# Autodesk Inventor assembly: Assembly1
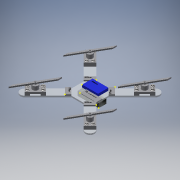
[picture p0: Inventor's stored thumbnail of the model, 180x180]
Saved by Autodesk Inventor 2019.4 (Build 234330000, 330)
## iProperties
Created: 2019-06-13
Part Number: Assembly1
Document SubType Name: Assembly
Designer: abdel
Author: abdel
## Documents named in this file (11)
- C:\Users\abdel\Downloads\10% project (laptop)-20190621T144919Z-001\10_ project (laptop)\drone\drone inventor\Assembly1.iam
- C:\Users\abdel\Downloads\10% project (laptop)-20190621T144919Z-001\10_ project (laptop)\drone\drone inventor\drone frame.ipt
- C:\Users\abdel\Downloads\10% project (laptop)-20190621T144919Z-001\10_ project (laptop)\drone\drone inventor\MotorController.ipt
- C:\Users\abdel\Downloads\10% project (laptop)-20190621T144919Z-001\10_ project (laptop)\drone\drone inventor\BracketOfTheBracket.ipt
- C:\Users\abdel\Downloads\10% project (laptop)-20190621T144919Z-001\10_ project (laptop)\drone\drone inventor\bracket for drone.ipt
- C:\Users\abdel\Downloads\10% project (laptop)-20190621T144919Z-001\10_ project (laptop)\drone\drone inventor\Motor.ipt
- C:\Users\abdel\Downloads\10% project (laptop)-20190621T144919Z-001\10_ project (laptop)\drone\drone inventor\Propeller.ipt
- C:\Users\abdel\Downloads\10% project (laptop)-20190621T144919Z-001\10_ project (laptop)\drone\drone inventor\battery.ipt
- C:\Users\abdel\Downloads\10% project (laptop)-20190621T144919Z-001\10_ project (laptop)\drone\drone inventor\GyroSensor.ipt
- C:\Users\abdel\Documents\Inventor\Content Center Files\R2019\en-US\GB_T 16674.1-2004\Bolt GB_T 16674.1 M8 x 16.ipt
- C:\Users\abdel\Downloads\10% project (laptop)-20190621T144919Z-001\10_ project (laptop)\drone\drone inventor\Arduino.ipt
## Components (44 placed, 10 different names)
1. battery:1 — Mate:41, Flush:24
2. bracket for drone:1 — Flush:3, Flush:4, Mate:4, Flush:5, Flush:6, Mate:5, Mate:6, Mate:7, Flush:11, Mate:42, Mate:43, Mate:44, Mate:45, Mate:46, Mate:47, Mate:48, Mate:49
3. drone frame:1 — Mate:12, Mate:13, Flush:11, Mate:18, Mate:19, Flush:16, Mate:24, Mate:25, Flush:21, Mate:26, Mate:27, Flush:22, Mate:28, Mate:29, Mate:30, Mate:31, Mate:32, Mate:33, Mate:34, Mate:35, Mate:36, Mate:37, Mate:38, Mate:39, Mate:40, Flush:23, Mate:41, Flush:24, Mate:66
4. Motor:1 — Rotational:1, Mate:6, Mate:7
5. MotorController:1 — Mate:28, Mate:29, Mate:30
6. Propeller:1 — Rotational:1
7. BracketOfTheBracket:3 — Flush:5, Flush:6, Mate:5
8. BracketOfTheBracket:5 — Flush:3, Flush:4, Mate:4, Mate:12, Mate:13
9. bracket for drone:2 — Flush:22, Mate:58, Mate:59, Mate:60, Mate:61, Mate:62, Mate:63, Mate:64, Mate:65
10. Motor:2
11. Propeller:2
12. BracketOfTheBracket:6
13. BracketOfTheBracket:7 — Mate:26, Mate:27
14. bracket for drone:3 — Flush:16, Mate:50, Mate:51, Mate:52, Mate:53, Mate:54, Mate:55, Mate:56, Mate:57
15. Motor:3
16. Propeller:3
17. BracketOfTheBracket:8
18. BracketOfTheBracket:9 — Mate:18, Mate:19
19. bracket for drone:4 — Flush:21, Insert:1, Insert:2, Insert:3, Insert:4
20. Motor:4
21. Propeller:4
22. BracketOfTheBracket:10 — Mate:25
23. BracketOfTheBracket:11 — Mate:24
24. MotorController:2 — Mate:31, Mate:32, Mate:33
25. MotorController:3 — Mate:34, Mate:35, Mate:36
26. MotorController:4 — Mate:37, Mate:38, Mate:39
27. GyroSensor:1 — Mate:40, Flush:23
28. Bolt GB/T 16674.1-2004 M8x16:1 — Insert:1
29. Bolt GB/T 16674.1-2004 M8x16:2 — Insert:2
30. Bolt GB/T 16674.1-2004 M8x16:3 — Insert:3
31. Bolt GB/T 16674.1-2004 M8x16:4 — Insert:4
32. Bolt GB/T 16674.1-2004 M8x16:5 — Mate:42, Mate:43
33. Bolt GB/T 16674.1-2004 M8x16:6 — Mate:44, Mate:45
34. Bolt GB/T 16674.1-2004 M8x16:7 — Mate:46, Mate:47
35. Bolt GB/T 16674.1-2004 M8x16:8 — Mate:48, Mate:49
36. Bolt GB/T 16674.1-2004 M8x16:9 — Mate:50, Mate:51
37. Bolt GB/T 16674.1-2004 M8x16:10 — Mate:52, Mate:53
38. Bolt GB/T 16674.1-2004 M8x16:11 — Mate:54, Mate:55
39. Bolt GB/T 16674.1-2004 M8x16:12 — Mate:56, Mate:57
40. Bolt GB/T 16674.1-2004 M8x16:13 — Mate:58, Mate:59
41. Bolt GB/T 16674.1-2004 M8x16:14 — Mate:60, Mate:61
42. Bolt GB/T 16674.1-2004 M8x16:15 — Mate:62, Mate:63
43. Bolt GB/T 16674.1-2004 M8x16:16 — Mate:64, Mate:65
44. Arduino:1 — Mate:66
## Relationships (93: Mate 63, Flush 22, RevoluteJoint 4, Insert 4)
- Rotational:1 [RevoluteJoint]: Motor:1 ↔ Propeller:1
- Flush:3: bracket for drone:1 ↔ BracketOfTheBracket:5
- Flush:4: bracket for drone:1 ↔ BracketOfTheBracket:5
- Mate:4: bracket for drone:1 ↔ BracketOfTheBracket:5
- Flush:5: bracket for drone:1 ↔ BracketOfTheBracket:3
- Flush:6: bracket for drone:1 ↔ BracketOfTheBracket:3
- Mate:5: bracket for drone:1 ↔ BracketOfTheBracket:3
- Mate:6: bracket for drone:1 ↔ Motor:1
- Mate:7: bracket for drone:1 ↔ Motor:1
- [RevoluteJoint]: Motor:2 ↔ Propeller:2
- [Flush]: bracket for drone:2 ↔ BracketOfTheBracket:7
- [Flush]: bracket for drone:2 ↔ BracketOfTheBracket:7
- [Mate]: bracket for drone:2 ↔ BracketOfTheBracket:7
- [Flush]: bracket for drone:2 ↔ BracketOfTheBracket:6
- [Flush]: bracket for drone:2 ↔ BracketOfTheBracket:6
- [Mate]: bracket for drone:2 ↔ BracketOfTheBracket:6
- [Mate]: bracket for drone:2 ↔ Motor:2
- [Mate]: bracket for drone:2 ↔ Motor:2
- Mate:12: drone frame:1 ↔ BracketOfTheBracket:5
- Mate:13: drone frame:1 ↔ BracketOfTheBracket:5
- Flush:11: bracket for drone:1 ↔ drone frame:1
- [RevoluteJoint]: Motor:3 ↔ Propeller:3
- [Flush]: bracket for drone:3 ↔ BracketOfTheBracket:9
- [Flush]: bracket for drone:3 ↔ BracketOfTheBracket:9
- [Mate]: bracket for drone:3 ↔ BracketOfTheBracket:9
- [Flush]: bracket for drone:3 ↔ BracketOfTheBracket:8
- [Flush]: bracket for drone:3 ↔ BracketOfTheBracket:8
- [Mate]: bracket for drone:3 ↔ BracketOfTheBracket:8
- [Mate]: bracket for drone:3 ↔ Motor:3
- [Mate]: bracket for drone:3 ↔ Motor:3
- Mate:18: drone frame:1 ↔ BracketOfTheBracket:9
- Mate:19: drone frame:1 ↔ BracketOfTheBracket:9
- Flush:16: drone frame:1 ↔ bracket for drone:3
- [RevoluteJoint]: Motor:4 ↔ Propeller:4
- [Flush]: bracket for drone:4 ↔ BracketOfTheBracket:11
- [Flush]: bracket for drone:4 ↔ BracketOfTheBracket:11
- [Mate]: bracket for drone:4 ↔ BracketOfTheBracket:11
- [Flush]: bracket for drone:4 ↔ BracketOfTheBracket:10
- [Flush]: bracket for drone:4 ↔ BracketOfTheBracket:10
- [Mate]: bracket for drone:4 ↔ BracketOfTheBracket:10
- [Mate]: bracket for drone:4 ↔ Motor:4
- [Mate]: bracket for drone:4 ↔ Motor:4
- Mate:24: drone frame:1 ↔ BracketOfTheBracket:11
- Mate:25: drone frame:1 ↔ BracketOfTheBracket:10
- Flush:21: drone frame:1 ↔ bracket for drone:4
- Mate:26: drone frame:1 ↔ BracketOfTheBracket:7
- Mate:27: drone frame:1 ↔ BracketOfTheBracket:7
- Flush:22: drone frame:1 ↔ bracket for drone:2
- Mate:28: drone frame:1 ↔ MotorController:1
- Mate:29: drone frame:1 ↔ MotorController:1
- Mate:30: drone frame:1 ↔ MotorController:1
- Mate:31: drone frame:1 ↔ MotorController:2
- Mate:32: drone frame:1 ↔ MotorController:2
- Mate:33: drone frame:1 ↔ MotorController:2
- Mate:34: drone frame:1 ↔ MotorController:3
- Mate:35: drone frame:1 ↔ MotorController:3
- Mate:36: drone frame:1 ↔ MotorController:3
- Mate:37: drone frame:1 ↔ MotorController:4
- Mate:38: drone frame:1 ↔ MotorController:4
- Mate:39: drone frame:1 ↔ MotorController:4
- Mate:40: drone frame:1 ↔ GyroSensor:1
- Flush:23: drone frame:1 ↔ GyroSensor:1
- Mate:41: battery:1 ↔ drone frame:1
- Flush:24: battery:1 ↔ drone frame:1
- Insert:1: bracket for drone:4 ↔ Bolt GB/T 16674.1-2004 M8x16:1
- Insert:2: bracket for drone:4 ↔ Bolt GB/T 16674.1-2004 M8x16:2
- Insert:3: bracket for drone:4 ↔ Bolt GB/T 16674.1-2004 M8x16:3
- Insert:4: bracket for drone:4 ↔ Bolt GB/T 16674.1-2004 M8x16:4
- Mate:42: bracket for drone:1 ↔ Bolt GB/T 16674.1-2004 M8x16:5
- Mate:43: bracket for drone:1 ↔ Bolt GB/T 16674.1-2004 M8x16:5
- Mate:44: bracket for drone:1 ↔ Bolt GB/T 16674.1-2004 M8x16:6
- Mate:45: bracket for drone:1 ↔ Bolt GB/T 16674.1-2004 M8x16:6
- Mate:46: bracket for drone:1 ↔ Bolt GB/T 16674.1-2004 M8x16:7
- Mate:47: bracket for drone:1 ↔ Bolt GB/T 16674.1-2004 M8x16:7
- Mate:48: bracket for drone:1 ↔ Bolt GB/T 16674.1-2004 M8x16:8
- Mate:49: bracket for drone:1 ↔ Bolt GB/T 16674.1-2004 M8x16:8
- Mate:50: bracket for drone:3 ↔ Bolt GB/T 16674.1-2004 M8x16:9
- Mate:51: bracket for drone:3 ↔ Bolt GB/T 16674.1-2004 M8x16:9
- Mate:52: bracket for drone:3 ↔ Bolt GB/T 16674.1-2004 M8x16:10
- Mate:53: bracket for drone:3 ↔ Bolt GB/T 16674.1-2004 M8x16:10
- Mate:54: bracket for drone:3 ↔ Bolt GB/T 16674.1-2004 M8x16:11
- Mate:55: bracket for drone:3 ↔ Bolt GB/T 16674.1-2004 M8x16:11
- Mate:56: bracket for drone:3 ↔ Bolt GB/T 16674.1-2004 M8x16:12
- Mate:57: bracket for drone:3 ↔ Bolt GB/T 16674.1-2004 M8x16:12
- Mate:58: bracket for drone:2 ↔ Bolt GB/T 16674.1-2004 M8x16:13
- Mate:59: bracket for drone:2 ↔ Bolt GB/T 16674.1-2004 M8x16:13
- Mate:60: bracket for drone:2 ↔ Bolt GB/T 16674.1-2004 M8x16:14
- Mate:61: bracket for drone:2 ↔ Bolt GB/T 16674.1-2004 M8x16:14
- Mate:62: bracket for drone:2 ↔ Bolt GB/T 16674.1-2004 M8x16:15
- Mate:63: bracket for drone:2 ↔ Bolt GB/T 16674.1-2004 M8x16:15
- Mate:64: bracket for drone:2 ↔ Bolt GB/T 16674.1-2004 M8x16:16
- Mate:65: bracket for drone:2 ↔ Bolt GB/T 16674.1-2004 M8x16:16
- Mate:66: drone frame:1 ↔ Arduino:1
## Named parameters: d74_d73 = 0 mm, d75_d66 = 0 mm, d76_d67 = 0 mm, d77_d68 = 0 mm, d78_d69 = 0 mm, d79_d70 = 0 mm, d80_d71 = 0 mm, d81_d72 = 0 mm, d82_d59 = 0 mm, d83_d60 = 0 deg, d87_d74_d73 = 0 mm, d88_d75_d66 = 0 mm, d89_d76_d67 = 0 mm, d90_d77_d68 = 0 mm, d91_d78_d69 = 0 mm, d92_d79_d70 = 0 mm, d93_d80_d71 = 0 mm, d94_d81_d72 = 0 mm, d95_d82_d59 = 0 mm, d96_d83_d60 = 0 deg, d100_d74_d73 = 0 mm, d101_d75_d66 = 0 mm, d102_d76_d67 = 0 mm, d103_d77_d68 = 0 mm, d104_d78_d69 = 0 mm, d105_d79_d70 = 0 mm, d106_d80_d71 = 0 mm, d107_d81_d72 = 0 mm, d108_d82_d59 = 0 mm, d109_d83_d60 = 0 deg
